# Autodesk Inventor assembly: Assembly1
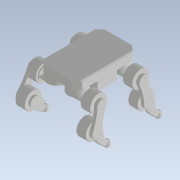
[picture p0: Inventor's stored thumbnail of the model, 180x180]
Saved by Autodesk Inventor 2020 (Build 240168000, 168)
## iProperties
Created: 2020-12-20
Part Number: Assembly1
Document SubType Name: Assembly
Designer: DELL
Author: DELL
## Documents named in this file (7)
- F:\SoftRobot2.0\12Dof\Assembly1.iam
- F:\SoftRobot2.0\Leg_Model\body_5.ipt
- F:\SoftRobot2.0\Leg_Model\connect_board5.ipt
- F:\SoftRobot2.0\Leg_Model\leg_demo_8.ipt
- F:\SoftRobot2.0\Leg_Model\connect_board4.ipt
- F:\SoftRobot2.0\Leg_Model\leg_demo_9.ipt
- F:\SoftRobot2.0\Leg_Model\RMD-X6.ipt
## Components (29 placed, 6 different names)
1. body_5:1 — Flush:1, Mate:3, Flush:5, Mate:89, Mate:90, Mate:91, Mate:92, Mate:104, Mate:105, Mate:110, Mate:111
2. RMD-X6:1 — Mate:30, Mate:31, Mate:46, Mate:47
3. connect_board5:3 — Mate:64, Mate:66, Mate:93, Mate:94
4. connect_board5:4 — Mate:56, Mate:57, Mate:87, Mate:88
5. leg_demo_8:1 — Mate:30, Mate:31, Mate:58, Mate:59
6. leg_demo_8:2 — Mate:63, Mate:65, Mate:95, Mate:103
7. leg_demo_8:3 — Mate:67, Mate:69, Mate:70, Mate:72
8. leg_demo_8:4 — Mate:73, Mate:75, Mate:76, Mate:79, Mate:80
9. connect_board4:1 — Mate:52, Tangent:1, Flush:6, Mate:78, Mate:81, Mate:101
10. connect_board4:2 — Flush:7, Mate:53, Tangent:2, Mate:71, Mate:82
11. connect_board4:3 — Mate:55, Flush:9, Tangent:4, Mate:60, Mate:61, Mate:62
12. connect_board4:4 — Mate:46, Mate:47, Mate:54, Flush:8, Tangent:3
13. leg_demo_9:1 — Mate:52, Tangent:1, Flush:6
14. leg_demo_9:2 — Mate:54, Flush:8, Tangent:3
15. leg_demo_9:3 — Mate:55, Flush:9, Tangent:4
16. leg_demo_9:4 — Flush:7, Mate:53, Tangent:2
17. RMD-X6:2 — Mate:56, Mate:57, Mate:58, Mate:59
18. RMD-X6:3 — Mate:64, Mate:65, Mate:66, Mate:95
19. RMD-X6:4 — Mate:60, Mate:61, Mate:62, Mate:63, Mate:103
20. RMD-X6:5 — Mate:67, Mate:69, Mate:114, Mate:115
21. RMD-X6:6 — Mate:70, Mate:71, Mate:72, Mate:82
22. RMD-X6:7 — Mate:78, Mate:79, Mate:80, Mate:81, Mate:101
23. RMD-X6:8 — Mate:73, Mate:75, Mate:76, Mate:108, Mate:109
24. RMD-X6:10 — Mate:87, Mate:88, Mate:89, Mate:90
25. RMD-X6:11 — Mate:91, Mate:92, Mate:93, Mate:94
26. RMD-X6:13 — Mate:104, Mate:105, Mate:106, Mate:107
27. connect_board5:5 — Mate:106, Mate:107, Mate:108, Mate:109
28. RMD-X6:14 — Mate:110, Mate:111, Mate:112, Mate:113
29. connect_board5:6 — Mate:112, Mate:113, Mate:114, Mate:115
## Relationships (66: Mate 56, Flush 6, Tangent 4)
- Flush:1: body_5:1
- Mate:3: body_5:1
- Flush:5: body_5:1
- Mate:30: RMD-X6:1 ↔ leg_demo_8:1
- Mate:31: RMD-X6:1 ↔ leg_demo_8:1
- Mate:46: RMD-X6:1 ↔ connect_board4:4
- Mate:47: RMD-X6:1 ↔ connect_board4:4
- Mate:52: connect_board4:1 ↔ leg_demo_9:1
- Tangent:1: connect_board4:1 ↔ leg_demo_9:1
- Flush:6: connect_board4:1 ↔ leg_demo_9:1
- Flush:7: connect_board4:2 ↔ leg_demo_9:4
- Mate:53: connect_board4:2 ↔ leg_demo_9:4
- Tangent:2: connect_board4:2 ↔ leg_demo_9:4
- Mate:54: connect_board4:4 ↔ leg_demo_9:2
- Flush:8: connect_board4:4 ↔ leg_demo_9:2
- Tangent:3: connect_board4:4 ↔ leg_demo_9:2
- Mate:55: connect_board4:3 ↔ leg_demo_9:3
- Flush:9: connect_board4:3 ↔ leg_demo_9:3
- Tangent:4: connect_board4:3 ↔ leg_demo_9:3
- Mate:56: connect_board5:4 ↔ RMD-X6:2
- Mate:57: connect_board5:4 ↔ RMD-X6:2
- Mate:58: leg_demo_8:1 ↔ RMD-X6:2
- Mate:59: leg_demo_8:1 ↔ RMD-X6:2
- Mate:60: connect_board4:3 ↔ RMD-X6:4
- Mate:61: connect_board4:3 ↔ RMD-X6:4
- Mate:62: connect_board4:3 ↔ RMD-X6:4
- Mate:63: leg_demo_8:2 ↔ RMD-X6:4
- Mate:64: connect_board5:3 ↔ RMD-X6:3
- Mate:65: leg_demo_8:2 ↔ RMD-X6:3
- Mate:66: connect_board5:3 ↔ RMD-X6:3
- Mate:67: leg_demo_8:3 ↔ RMD-X6:5
- Mate:69: leg_demo_8:3 ↔ RMD-X6:5
- Mate:70: leg_demo_8:3 ↔ RMD-X6:6
- Mate:71: connect_board4:2 ↔ RMD-X6:6
- Mate:72: leg_demo_8:3 ↔ RMD-X6:6
- Mate:73: leg_demo_8:4 ↔ RMD-X6:8
- Mate:75: leg_demo_8:4 ↔ RMD-X6:8
- Mate:76: leg_demo_8:4 ↔ RMD-X6:8
- Mate:78: connect_board4:1 ↔ RMD-X6:7
- Mate:79: leg_demo_8:4 ↔ RMD-X6:7
- Mate:80: leg_demo_8:4 ↔ RMD-X6:7
- Mate:81: connect_board4:1 ↔ RMD-X6:7
- Mate:82: connect_board4:2 ↔ RMD-X6:6
- Mate:87: connect_board5:4 ↔ RMD-X6:10
- Mate:88: connect_board5:4 ↔ RMD-X6:10
- Mate:89: body_5:1 ↔ RMD-X6:10
- Mate:90: body_5:1 ↔ RMD-X6:10
- Mate:91: body_5:1 ↔ RMD-X6:11
- Mate:92: body_5:1 ↔ RMD-X6:11
- Mate:93: connect_board5:3 ↔ RMD-X6:11
- Mate:94: connect_board5:3 ↔ RMD-X6:11
- Mate:95: leg_demo_8:2 ↔ RMD-X6:3
- Mate:101: connect_board4:1 ↔ RMD-X6:7
- Mate:103: leg_demo_8:2 ↔ RMD-X6:4
- Mate:104: body_5:1 ↔ RMD-X6:13
- Mate:105: body_5:1 ↔ RMD-X6:13
- Mate:106: RMD-X6:13 ↔ connect_board5:5
- Mate:107: RMD-X6:13 ↔ connect_board5:5
- Mate:108: RMD-X6:8 ↔ connect_board5:5
- Mate:109: RMD-X6:8 ↔ connect_board5:5
- Mate:110: body_5:1 ↔ RMD-X6:14
- Mate:111: body_5:1 ↔ RMD-X6:14
- Mate:112: RMD-X6:14 ↔ connect_board5:6
- Mate:113: RMD-X6:14 ↔ connect_board5:6
- Mate:114: RMD-X6:5 ↔ connect_board5:6
- Mate:115: RMD-X6:5 ↔ connect_board5:6
